# Autodesk Inventor assembly: Сборка вала
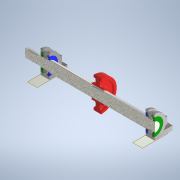
[picture p0: Inventor's stored thumbnail of the model, 180x180]
Saved by Autodesk Inventor 2021 (Build 250183000, 183)
## iProperties
Created: 2023-04-24
Part Number: Сборка вала
Document SubType Name: Assembly
Designer: gdevc
Author: gdevc
## Documents named in this file (9)
- C:\Users\gdevc\OneDrive\Рабочий стол\Курсач\DetaliMashine\Новая папка\Приводной валл\Сборка вала.iam
- C:\Users\gdevc\OneDrive\Рабочий стол\Курсач\DetaliMashine\Новая папка\Приводной валл\Валл.ipt
- C:\Users\gdevc\OneDrive\Рабочий стол\Курсач\DetaliMashine\Новая папка\Приводной валл\звездочка.ipt
- C:\Users\gdevc\OneDrive\Рабочий стол\Курсач\DetaliMashine\Новая папка\Приводной валл\Подшипник 1211 ГОСТ 28428-90.ipt
- C:\Users\gdevc\OneDrive\Рабочий стол\Курсач\DetaliMashine\Новая папка\Приводной валл\Манжет 2-55x72x8 ГОСТ 8752-79.ipt
- C:\Users\gdevc\OneDrive\Рабочий стол\Курсач\DetaliMashine\Новая папка\Приводной валл\Манжет 2-60x80x8 ГОСТ 8752-79.ipt
- C:\Users\gdevc\OneDrive\Рабочий стол\Курсач\DetaliMashine\Новая папка\Приводной валл\Крышка_Левая.ipt
- C:\Users\gdevc\OneDrive\Рабочий стол\Курсач\DetaliMashine\Новая папка\Приводной валл\Крышка правая.ipt
- C:\Users\gdevc\OneDrive\Рабочий стол\Курсач\DetaliMashine\Новая папка\Приводной валл\Корпус_Подшипника.ipt
## Components (14 placed, 8 different names)
1. Валл:1 — Совмещение:1, Совмещение:2, Совмещение:4, Совмещение:5, Совмещение:6, Совмещение:7, Совмещение:8, Совмещение:11, Совмещение:12, Совмещение:15, Совмещение:16, Совмещение:17, Совмещение:20, Совмещение:23, Совмещение:25, Заподлицо:1
2. звездочка:1 — Совмещение:1, Угол:1, Заподлицо:1
3. Подшипник 1211 ГОСТ 28428-90:1 — Совмещение:2, Совмещение:4, Угол:2, Совмещение:9, Совмещение:13
4. Подшипник 1211 ГОСТ 28428-90:2 — Совмещение:5, Совмещение:6, Совмещение:19, Совмещение:22
5. Манжет 2-55x72x8 ГОСТ 8752-79:1 — Совмещение:7, Совмещение:10
6. Манжет 2-60x80x8 ГОСТ 8752-79:1 — Совмещение:11, Совмещение:14
7. Крышка_Левая:1 — Совмещение:8, Совмещение:9, Совмещение:10, Совмещение:24
8. Крышка правая:1 — Совмещение:12, Совмещение:13, Совмещение:14
9. Крышка правая:2 — Совмещение:17, Совмещение:18, Совмещение:19, Совмещение:26
10. Крышка_Левая:2 — Совмещение:20, Совмещение:21, Совмещение:22
11. Манжет 2-55x72x8 ГОСТ 8752-79:2 — Совмещение:16, Совмещение:21
12. Манжет 2-60x80x8 ГОСТ 8752-79:2 — Совмещение:15, Совмещение:18
13. Корпус_Подшипника:1 — Совмещение:23, Угол:3, Совмещение:24
14. Корпус_Подшипника:2 — Угол:4, Совмещение:25, Совмещение:26
## Relationships (30: Mate 25, Angle 4, Flush 1)
- Совмещение:1 [Mate]: Валл:1 ↔ звездочка:1
- Угол:1 [Angle] (180 deg): звездочка:1
- Совмещение:2 [Mate]: Валл:1 ↔ Подшипник 1211 ГОСТ 28428-90:1
- Совмещение:4 [Mate]: Валл:1 ↔ Подшипник 1211 ГОСТ 28428-90:1
- Совмещение:5 [Mate]: Валл:1 ↔ Подшипник 1211 ГОСТ 28428-90:2
- Совмещение:6 [Mate]: Валл:1 ↔ Подшипник 1211 ГОСТ 28428-90:2
- Угол:2 [Angle] (0 deg): Подшипник 1211 ГОСТ 28428-90:1
- Совмещение:7 [Mate]: Валл:1 ↔ Манжет 2-55x72x8 ГОСТ 8752-79:1
- Совмещение:8 [Mate]: Валл:1 ↔ Крышка_Левая:1
- Совмещение:9 [Mate]: Подшипник 1211 ГОСТ 28428-90:1 ↔ Крышка_Левая:1
- Совмещение:10 [Mate]: Манжет 2-55x72x8 ГОСТ 8752-79:1 ↔ Крышка_Левая:1
- Совмещение:11 [Mate]: Валл:1 ↔ Манжет 2-60x80x8 ГОСТ 8752-79:1
- Совмещение:12 [Mate]: Валл:1 ↔ Крышка правая:1
- Совмещение:13 [Mate]: Подшипник 1211 ГОСТ 28428-90:1 ↔ Крышка правая:1
- Совмещение:14 [Mate]: Манжет 2-60x80x8 ГОСТ 8752-79:1 ↔ Крышка правая:1
- Совмещение:15 [Mate]: Валл:1 ↔ Манжет 2-60x80x8 ГОСТ 8752-79:2
- Совмещение:16 [Mate]: Валл:1 ↔ Манжет 2-55x72x8 ГОСТ 8752-79:2
- Совмещение:17 [Mate]: Валл:1 ↔ Крышка правая:2
- Совмещение:18 [Mate]: Крышка правая:2 ↔ Манжет 2-60x80x8 ГОСТ 8752-79:2
- Совмещение:19 [Mate]: Подшипник 1211 ГОСТ 28428-90:2 ↔ Крышка правая:2
- Совмещение:20 [Mate]: Валл:1 ↔ Крышка_Левая:2
- Совмещение:21 [Mate]: Крышка_Левая:2 ↔ Манжет 2-55x72x8 ГОСТ 8752-79:2
- Совмещение:22 [Mate]: Подшипник 1211 ГОСТ 28428-90:2 ↔ Крышка_Левая:2
- Совмещение:23 [Mate]: Валл:1 ↔ Корпус_Подшипника:1
- Угол:3 [Angle] (0 deg): Корпус_Подшипника:1
- Совмещение:24 [Mate]: Крышка_Левая:1 ↔ Корпус_Подшипника:1
- Угол:4 [Angle] (0 deg): Корпус_Подшипника:2
- Совмещение:25 [Mate]: Валл:1 ↔ Корпус_Подшипника:2
- Совмещение:26 [Mate]: Крышка правая:2 ↔ Корпус_Подшипника:2
- Заподлицо:1 [Flush] (242.5 mm): Валл:1 ↔ звездочка:1
